# Autodesk Inventor assembly: EnsambleHexapod
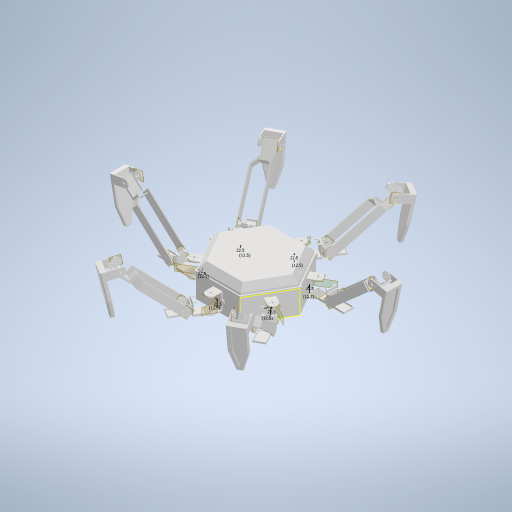
[picture p0: Inventor's stored thumbnail of the model, 512x512]
Saved by Autodesk Inventor 2024 (Build 280153000, 153)
## iProperties
Created: 2024-03-17
Part Number: EnsambleHexapod
Document SubType Name: Assembly
Designer: na_re
Author: na_re
## Documents named in this file (4)
- C:\Users\na_re\OneDrive\Escritorio\CAD_NAOMI\EnsambleHexapod.iam
- C:\Users\Public\Documents\Autodesk\Inventor 2024\HEXAPOD_CAD\BaseHEX.ipt
- C:\Users\Public\Documents\Autodesk\Inventor 2024\HEXAPOD_CAD\tapaHEX.ipt
- C:\Users\Public\Documents\Autodesk\Inventor 2024\Pata.iam
## Components (8 placed, 3 different names)
1. BaseHEX:1 — Nivelación:1, Nivelación:2, Coincidencia:1, Coincidencia:2, Coincidencia:3, Coincidencia:4, Coincidencia:5, Coincidencia:6, Coincidencia:7, Coincidencia:8, Coincidencia:9, Coincidencia:10, Coincidencia:11, Coincidencia:12, Coincidencia:13, Coincidencia:14, Coincidencia:15, Coincidencia:16, Coincidencia:17, Coincidencia:18
2. tapaHEX:1 — Nivelación:1, Nivelación:2
3. Pata:1 [sub-assembly] — Coincidencia:1, Coincidencia:2, Coincidencia:3
4. Pata:2 [sub-assembly] — Coincidencia:4, Coincidencia:5, Coincidencia:6
5. Pata:3 [sub-assembly] — Coincidencia:7, Coincidencia:8, Coincidencia:9
6. Pata:4 [sub-assembly] — Coincidencia:10, Coincidencia:11, Coincidencia:12
7. Pata:5 [sub-assembly] — Coincidencia:13, Coincidencia:14, Coincidencia:15
8. Pata:6 [sub-assembly] — Coincidencia:16, Coincidencia:17, Coincidencia:18
## Relationships (20: Mate 18, Flush 2)
- Nivelación:1 [Flush]: BaseHEX:1 ↔ tapaHEX:1
- Nivelación:2 [Flush]: BaseHEX:1 ↔ tapaHEX:1
- Coincidencia:1 [Mate]: BaseHEX:1 ↔ Pata:1
- Coincidencia:2 [Mate]: BaseHEX:1 ↔ Pata:1
- Coincidencia:3 [Mate]: BaseHEX:1 ↔ Pata:1
- Coincidencia:4 [Mate]: BaseHEX:1 ↔ Pata:2
- Coincidencia:5 [Mate]: BaseHEX:1 ↔ Pata:2
- Coincidencia:6 [Mate]: BaseHEX:1 ↔ Pata:2
- Coincidencia:7 [Mate]: BaseHEX:1 ↔ Pata:3
- Coincidencia:8 [Mate]: BaseHEX:1 ↔ Pata:3
- Coincidencia:9 [Mate]: BaseHEX:1 ↔ Pata:3
- Coincidencia:10 [Mate]: BaseHEX:1 ↔ Pata:4
- Coincidencia:11 [Mate]: BaseHEX:1 ↔ Pata:4
- Coincidencia:12 [Mate]: BaseHEX:1 ↔ Pata:4
- Coincidencia:13 [Mate]: BaseHEX:1 ↔ Pata:5
- Coincidencia:14 [Mate]: BaseHEX:1 ↔ Pata:5
- Coincidencia:15 [Mate]: BaseHEX:1 ↔ Pata:5
- Coincidencia:16 [Mate]: BaseHEX:1 ↔ Pata:6
- Coincidencia:17 [Mate]: BaseHEX:1 ↔ Pata:6
- Coincidencia:18 [Mate]: BaseHEX:1 ↔ Pata:6
